# Autodesk Inventor assembly: McCrea_RUKA_TELO_SPOJ_walle
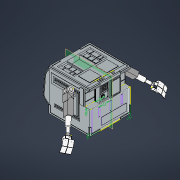
[picture p0: Inventor's stored thumbnail of the model, 180x180]
Saved by Autodesk Inventor 2022 (Build 260153000, 153)
## iProperties
Created: 2022-02-01
Part Number: McCrea_RUKA_TELO_SPOJ_walle
Document SubType Name: Assembly
Designer: MatusBarany
Author: MatusBarany
## Documents named in this file (4)
- C:\Users\MatusBarany\Documents\Inventor\wall-e\lukas\McCrea_RUKA_TELO_SPOJ_walle.iam
- C:\Users\MatusBarany\Documents\Inventor\wall-e\lukas\McCrea_BODY_walle.iam
- C:\Users\MatusBarany\Documents\Inventor\wall-e\lukas\McCrea_RUKA_Walle.iam
- C:\Users\MatusBarany\Documents\Inventor\wall-e\lukas\McCrea_RUKA_Walle_MIR.iam
## Components (3 placed, 3 different names)
1. McCrea_BODY_walle:1 [sub-assembly] — Mate:1, Mate:2
2. McCrea_RUKA_Walle:1 [sub-assembly] — Mate:1, Mate:2
3. McCrea_RUKA_Walle_MIR:1 [sub-assembly]
## Relationships (2: Mate 2)
- Mate:1: McCrea_BODY_walle:1 ↔ McCrea_RUKA_Walle:1
- Mate:2: McCrea_BODY_walle:1 ↔ McCrea_RUKA_Walle:1
